# Autodesk Inventor assembly: WheelWithHexHub
Saved by Autodesk Inventor 2016 (Build 200138000, 138)
## iProperties
Created: 2017-01-08
Part Number: WheelWithHexHub
Document SubType Name: Assembly
Designer: Dhruv
Author: Dhruv
## Documents named in this file (4)
- C:\Users\Dhruv\Desktop\MISC\FRC 2017\WheelWithHexHub.iam
- C:\Users\Dhruv\Desktop\MISC\FRC 2017\supporting_parts\4 in HiGrip Wheel.ipt
- C:\Users\Dhruv\Desktop\MISC\FRC 2017\supporting_parts\am-2568 500EX Hex Hub.ipt
- C:\Users\Dhruv\Desktop\MISC\FRC 2017\supporting_parts\93075A249_ZINC-PLATED STEEL HEX HEAD MACHINE SCREW.ipt
## Components (8 placed, 3 different names)
1. 4 in HiGrip Wheel:1
2. am-2568 500EX Hex Hub:1
3. 93075A249_ZINC-PLATED STEEL HEX HEAD MACHINE SCREW:1
4. 93075A249_ZINC-PLATED STEEL HEX HEAD MACHINE SCREW:2
5. 93075A249_ZINC-PLATED STEEL HEX HEAD MACHINE SCREW:3
6. 93075A249_ZINC-PLATED STEEL HEX HEAD MACHINE SCREW:4
7. 93075A249_ZINC-PLATED STEEL HEX HEAD MACHINE SCREW:5
8. 93075A249_ZINC-PLATED STEEL HEX HEAD MACHINE SCREW:6
## Relationships (14: Mate 13, Insert 1)
- [Insert]: 4 in HiGrip Wheel:1 ↔ am-2568 500EX Hex Hub:1
- [Mate]: 4 in HiGrip Wheel:1 ↔ am-2568 500EX Hex Hub:1
- [Mate]: 4 in HiGrip Wheel:1 ↔ 93075A249_ZINC-PLATED STEEL HEX HEAD MACHINE SCREW:1
- [Mate]: am-2568 500EX Hex Hub:1 ↔ 93075A249_ZINC-PLATED STEEL HEX HEAD MACHINE SCREW:1
- [Mate]: am-2568 500EX Hex Hub:1 ↔ 93075A249_ZINC-PLATED STEEL HEX HEAD MACHINE SCREW:2
- [Mate]: am-2568 500EX Hex Hub:1 ↔ 93075A249_ZINC-PLATED STEEL HEX HEAD MACHINE SCREW:2
- [Mate]: am-2568 500EX Hex Hub:1 ↔ 93075A249_ZINC-PLATED STEEL HEX HEAD MACHINE SCREW:4
- [Mate]: am-2568 500EX Hex Hub:1 ↔ 93075A249_ZINC-PLATED STEEL HEX HEAD MACHINE SCREW:4
- [Mate]: am-2568 500EX Hex Hub:1 ↔ 93075A249_ZINC-PLATED STEEL HEX HEAD MACHINE SCREW:5
- [Mate]: am-2568 500EX Hex Hub:1 ↔ 93075A249_ZINC-PLATED STEEL HEX HEAD MACHINE SCREW:5
- [Mate]: am-2568 500EX Hex Hub:1 ↔ 93075A249_ZINC-PLATED STEEL HEX HEAD MACHINE SCREW:3
- [Mate]: am-2568 500EX Hex Hub:1 ↔ 93075A249_ZINC-PLATED STEEL HEX HEAD MACHINE SCREW:3
- [Mate]: am-2568 500EX Hex Hub:1 ↔ 93075A249_ZINC-PLATED STEEL HEX HEAD MACHINE SCREW:6
- [Mate]: am-2568 500EX Hex Hub:1 ↔ 93075A249_ZINC-PLATED STEEL HEX HEAD MACHINE SCREW:6
## Named parameters: d1_d12 = 0 mm, d2_d13 = 0 mm
